# Autodesk Inventor assembly: keywell
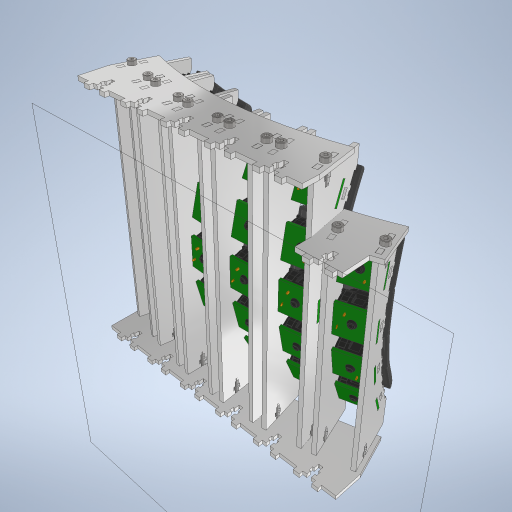
[picture p0: Inventor's stored thumbnail of the model, 512x512]
Saved by Autodesk Inventor 2024.1 (Build 281209000, 209)
## iProperties
Created: 2019-07-06
Part Number: keywell
Document SubType Name: Assembly
Designer: Thibault
Mass: 341.563 g
Surface Area: 1996.11 cm^2
Volume: 92.7912 cm^3
Density: 3.68098 g/cm^3
Author: Thibault
## Documents named in this file (14)
- C:\Users\Thibault\Documents\habilis\mech\keywell.iam
- C:\Users\Thibault\Documents\habilis\mech\switchplate\switchplate-1.iam
- C:\Users\Thibault Polge\Documents\Habilis\mech\switchplate.iam
- C:\Users\Thibault\Documents\habilis\mech\switchplate\switchplate-2.iam
- C:\Users\Thibault\Documents\habilis\mech\switchplate\switchplate-3.iam
- C:\Users\Thibault\Documents\habilis\mech\switchplate\switchplate-4.iam
- C:\Users\Thibault\Documents\habilis\mech\switchplate\switchplate-5.iam
- C:\Users\Thibault\Documents\habilis\mech\switchplate\switchplate-6.iam
- C:\Users\Thibault\Documents\habilis\mech\keywell_support\keywell_support-back.ipt
- C:\Users\Thibault Polge\Documents\Habilis\mech\keywell_support.ipt
- C:\Users\Thibault\Documents\habilis\mech\keywell_support\keywell_support-front.ipt
- C:\Users\Thibault\Documents\habilis\mech\keywell_support\keywell_support-front-r6.ipt
- C:\Users\Thibault\Documents\habilis\mech\shared_parameters.ipt
- C:\Users\Thibault\Documents\Inventor\Content Center Files\R2024\fr-FR\BS 4168(1)\BS 4168 - M2 x 10(1).ipt
## Components (33 placed, 10 different names)
1. keywell_support-back:1 — Affleurement:1, Affleurement:3, Affleurement:4, Affleurement:5, Affleurement:6, Affleurement:9, Placage:1, Placage:2, Placage:3, Placage:4, Placage:5, Placage:6, Placage:7, Placage:8, Placage:9, Placage:10, Placage:11, Placage:12, Affleurement:11
2. switchplate-1:1 [sub-assembly] — Affleurement:1, Affleurement:7, Placage:1, Placage:12
3. switchplate-2:2 [sub-assembly] — Affleurement:9, Placage:2, Placage:11
4. switchplate-3:3 [sub-assembly] — Affleurement:3, Placage:3, Placage:10
5. switchplate-4:4 [sub-assembly] — Affleurement:4, Placage:4, Placage:9
6. switchplate-5:5 [sub-assembly] — Affleurement:5, Placage:5, Placage:8
7. switchplate-6:6 [sub-assembly] — Affleurement:6, Placage:6, Placage:7, Affleurement:10, Placage:13, Placage:14
8. keywell_support-front:2 — Affleurement:7, Affleurement:11
9. keywell_support-front-r6:3 — Affleurement:10, Placage:13, Placage:14
10. BS 4168 : Pièce 1 Vis cylindrique à six pans creux - Métrique M2 x 10:1
11. BS 4168 : Pièce 1 Vis cylindrique à six pans creux - Métrique M2 x 10:2
12. BS 4168 : Pièce 1 Vis cylindrique à six pans creux - Métrique M2 x 10:3
13. BS 4168 : Pièce 1 Vis cylindrique à six pans creux - Métrique M2 x 10:4
14. BS 4168 : Pièce 1 Vis cylindrique à six pans creux - Métrique M2 x 10:5
15. BS 4168 : Pièce 1 Vis cylindrique à six pans creux - Métrique M2 x 10:6
16. BS 4168 : Pièce 1 Vis cylindrique à six pans creux - Métrique M2 x 10:7
17. BS 4168 : Pièce 1 Vis cylindrique à six pans creux - Métrique M2 x 10:8
18. BS 4168 : Pièce 1 Vis cylindrique à six pans creux - Métrique M2 x 10:9
19. BS 4168 : Pièce 1 Vis cylindrique à six pans creux - Métrique M2 x 10:10
20. BS 4168 : Pièce 1 Vis cylindrique à six pans creux - Métrique M2 x 10:11
21. BS 4168 : Pièce 1 Vis cylindrique à six pans creux - Métrique M2 x 10:12
22. BS 4168 : Pièce 1 Vis cylindrique à six pans creux - Métrique M2 x 10:13
23. BS 4168 : Pièce 1 Vis cylindrique à six pans creux - Métrique M2 x 10:14
24. BS 4168 : Pièce 1 Vis cylindrique à six pans creux - Métrique M2 x 10:15
25. BS 4168 : Pièce 1 Vis cylindrique à six pans creux - Métrique M2 x 10:16
26. BS 4168 : Pièce 1 Vis cylindrique à six pans creux - Métrique M2 x 10:17
27. BS 4168 : Pièce 1 Vis cylindrique à six pans creux - Métrique M2 x 10:18
28. BS 4168 : Pièce 1 Vis cylindrique à six pans creux - Métrique M2 x 10:19
29. BS 4168 : Pièce 1 Vis cylindrique à six pans creux - Métrique M2 x 10:20
30. BS 4168 : Pièce 1 Vis cylindrique à six pans creux - Métrique M2 x 10:21
31. BS 4168 : Pièce 1 Vis cylindrique à six pans creux - Métrique M2 x 10:22
32. BS 4168 : Pièce 1 Vis cylindrique à six pans creux - Métrique M2 x 10:23
33. BS 4168 : Pièce 1 Vis cylindrique à six pans creux - Métrique M2 x 10:24
## Relationships (47: Insert 24, Mate 14, Flush 9)
- Affleurement:1 [Flush]: keywell_support-back:1 ↔ switchplate-1:1
- Affleurement:3 [Flush]: keywell_support-back:1 ↔ switchplate-3:3
- Affleurement:4 [Flush]: keywell_support-back:1 ↔ switchplate-4:4
- Affleurement:5 [Flush]: keywell_support-back:1 ↔ switchplate-5:5
- Affleurement:6 [Flush]: keywell_support-back:1 ↔ switchplate-6:6
- Affleurement:7 [Flush]: switchplate-1:1 ↔ keywell_support-front:2
- Affleurement:9 [Flush]: keywell_support-back:1 ↔ switchplate-2:2
- [Insert]: keywell_support-front:2 ↔ BS 4168 : Pièce 1 Vis cylindrique à six pans creux - Métrique M2 x 10:1
- [Insert]: keywell_support-front:2 ↔ BS 4168 : Pièce 1 Vis cylindrique à six pans creux - Métrique M2 x 10:2
- [Insert]: keywell_support-front:2 ↔ BS 4168 : Pièce 1 Vis cylindrique à six pans creux - Métrique M2 x 10:3
- [Insert]: keywell_support-front:2 ↔ BS 4168 : Pièce 1 Vis cylindrique à six pans creux - Métrique M2 x 10:4
- [Insert]: keywell_support-front:2 ↔ BS 4168 : Pièce 1 Vis cylindrique à six pans creux - Métrique M2 x 10:5
- [Insert]: keywell_support-front:2 ↔ BS 4168 : Pièce 1 Vis cylindrique à six pans creux - Métrique M2 x 10:6
- [Insert]: keywell_support-front:2 ↔ BS 4168 : Pièce 1 Vis cylindrique à six pans creux - Métrique M2 x 10:7
- [Insert]: keywell_support-front:2 ↔ BS 4168 : Pièce 1 Vis cylindrique à six pans creux - Métrique M2 x 10:8
- [Insert]: keywell_support-front:2 ↔ BS 4168 : Pièce 1 Vis cylindrique à six pans creux - Métrique M2 x 10:9
- [Insert]: keywell_support-front:2 ↔ BS 4168 : Pièce 1 Vis cylindrique à six pans creux - Métrique M2 x 10:10
- [Insert]: keywell_support-front-r6:3 ↔ BS 4168 : Pièce 1 Vis cylindrique à six pans creux - Métrique M2 x 10:11
- [Insert]: keywell_support-front-r6:3 ↔ BS 4168 : Pièce 1 Vis cylindrique à six pans creux - Métrique M2 x 10:12
- [Insert]: keywell_support-back:1 ↔ BS 4168 : Pièce 1 Vis cylindrique à six pans creux - Métrique M2 x 10:13
- [Insert]: keywell_support-back:1 ↔ BS 4168 : Pièce 1 Vis cylindrique à six pans creux - Métrique M2 x 10:14
- [Insert]: keywell_support-back:1 ↔ BS 4168 : Pièce 1 Vis cylindrique à six pans creux - Métrique M2 x 10:15
- [Insert]: keywell_support-back:1 ↔ BS 4168 : Pièce 1 Vis cylindrique à six pans creux - Métrique M2 x 10:16
- [Insert]: keywell_support-back:1 ↔ BS 4168 : Pièce 1 Vis cylindrique à six pans creux - Métrique M2 x 10:17
- [Insert]: keywell_support-back:1 ↔ BS 4168 : Pièce 1 Vis cylindrique à six pans creux - Métrique M2 x 10:18
- [Insert]: keywell_support-back:1 ↔ BS 4168 : Pièce 1 Vis cylindrique à six pans creux - Métrique M2 x 10:19
- [Insert]: keywell_support-back:1 ↔ BS 4168 : Pièce 1 Vis cylindrique à six pans creux - Métrique M2 x 10:20
- [Insert]: keywell_support-back:1 ↔ BS 4168 : Pièce 1 Vis cylindrique à six pans creux - Métrique M2 x 10:21
- [Insert]: keywell_support-back:1 ↔ BS 4168 : Pièce 1 Vis cylindrique à six pans creux - Métrique M2 x 10:22
- [Insert]: keywell_support-back:1 ↔ BS 4168 : Pièce 1 Vis cylindrique à six pans creux - Métrique M2 x 10:23
- [Insert]: keywell_support-back:1 ↔ BS 4168 : Pièce 1 Vis cylindrique à six pans creux - Métrique M2 x 10:24
- Placage:1 [Mate]: keywell_support-back:1 ↔ switchplate-1:1
- Placage:2 [Mate]: keywell_support-back:1 ↔ switchplate-2:2
- Placage:3 [Mate]: keywell_support-back:1 ↔ switchplate-3:3
- Placage:4 [Mate]: keywell_support-back:1 ↔ switchplate-4:4
- Placage:5 [Mate]: keywell_support-back:1 ↔ switchplate-5:5
- Placage:6 [Mate]: keywell_support-back:1 ↔ switchplate-6:6
- Placage:7 [Mate]: keywell_support-back:1 ↔ switchplate-6:6
- Placage:8 [Mate]: keywell_support-back:1 ↔ switchplate-5:5
- Placage:9 [Mate]: keywell_support-back:1 ↔ switchplate-4:4
- Placage:10 [Mate]: keywell_support-back:1 ↔ switchplate-3:3
- Placage:11 [Mate]: keywell_support-back:1 ↔ switchplate-2:2
- Placage:12 [Mate]: keywell_support-back:1 ↔ switchplate-1:1
- Affleurement:10 [Flush]: switchplate-6:6 ↔ keywell_support-front-r6:3
- Placage:13 [Mate]: switchplate-6:6 ↔ keywell_support-front-r6:3
- Placage:14 [Mate]: switchplate-6:6 ↔ keywell_support-front-r6:3
- Affleurement:11 [Flush]: keywell_support-back:1 ↔ keywell_support-front:2
## Named parameters: extra_slot_dim = 0 mm
